# Autodesk Inventor assembly: 期末專案
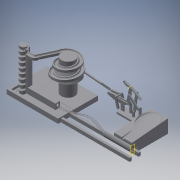
[picture p0: Inventor's stored thumbnail of the model, 180x180]
Saved by Autodesk Inventor 2017 (Build 210142000, 142)
## iProperties
Part Number: 期末專案
Material: 一般
Document SubType Name: Assembly
Designer: 士正
Author: 士正
## Documents named in this file (15)
- C:\Users\士正\Desktop\git\期末專案\期末專案.iam
- C:\Users\士正\Desktop\git\期末專案\實體1_3.ipt
- C:\Users\士正\Desktop\git\期末專案\實體2_3.ipt
- C:\Users\士正\Desktop\git\期末專案\實體3_3.ipt
- C:\Users\士正\Desktop\git\期末專案\實體4_3.ipt
- C:\Users\士正\Desktop\git\期末專案\實體5_3.ipt
- C:\Users\士正\Desktop\git\期末專案\實體6_3.ipt
- C:\Users\士正\Desktop\git\期末專案\實體7_3.ipt
- C:\Users\士正\Desktop\git\期末專案\實體8_3.ipt
- C:\Users\士正\Desktop\git\期末專案\實體9_3.ipt
- C:\Users\士正\Desktop\git\期末專案\實體10_2.ipt
- C:\Users\士正\Desktop\git\期末專案\實體11_2.ipt
- C:\Users\士正\Desktop\git\期末專案\螺旋5.ipt
- C:\Users\士正\Desktop\git\期末專案\零件2.ipt
- C:\Users\士正\Desktop\git\期末專案\長方形塊.ipt
## Components (28 placed, 14 different names)
1. 實體1_3:1 — 貼合:7, 貼合:8, 貼合:12
2. 實體2_3:1 — 貼合:11, 貼合:21, 貼合:22, 貼合:35, 齊平:11, 貼合:36, 齊平:12
3. 實體3_3:1 — 貼合:9, 貼合:10, 貼合:13, 貼合:14, 貼合:34, 齊平:10
4. 實體4_3:1 — 貼合:3, 貼合:4, 貼合:5, 貼合:6
5. 實體5_3:1 — 貼合:5, 貼合:6, 貼合:18, 貼合:29, 齊平:5
6. 實體6_3:1 — 貼合:1, 貼合:2, 貼合:17, 貼合:27, 齊平:3, 貼合:31, 齊平:7
7. 實體7_3:1 — 貼合:19, 貼合:20, 貼合:21, 貼合:22, 貼合:23, 貼合:25, 齊平:1, 貼合:37, 齊平:13, 貼合:40, 齊平:16
8. 實體8_3:1 — 貼合:12, 貼合:13, 貼合:14, 貼合:15, 貼合:16, 貼合:19, 貼合:20, 貼合:32, 齊平:8, 貼合:33, 齊平:9
9. 實體9_3:1 — 貼合:15, 貼合:16, 貼合:17, 貼合:18, 貼合:30, 齊平:6
10. 實體10_2:1 — 貼合:29, 齊平:5
11. 實體11_2:1 — 貼合:1, 貼合:2, 貼合:3, 貼合:4, 貼合:7, 貼合:8, 貼合:9, 貼合:10, 貼合:11, 貼合:24, 齊平:2, 貼合:26, 貼合:28, 齊平:4, 貼合:41, 齊平:17, 齊平:18
12. 實體2_3:2 — 貼合:23, 貼合:24, 貼合:25, 貼合:38, 齊平:14, 貼合:39, 齊平:15
13. 實體10_2:2 — 貼合:31, 齊平:7
14. 實體10_2:3 — 貼合:37, 齊平:13
15. 實體10_2:4 — 貼合:40, 齊平:16
16. 實體10_2:5 — 貼合:39, 齊平:15
17. 實體10_2:6 — 貼合:36, 齊平:12
18. 實體10_2:7 — 貼合:35, 齊平:11
19. 實體10_2:8 — 貼合:38, 齊平:14
20. 實體10_2:9 — 貼合:32, 齊平:8
21. 實體10_2:10 — 貼合:34, 齊平:10
22. 實體10_2:11 — 貼合:33, 齊平:9
23. 實體10_2:12 — 貼合:27, 齊平:3
24. 實體10_2:13 — 貼合:30, 齊平:6
25. 實體10_2:14 — 貼合:28, 齊平:4
26. 螺旋5:1 — 齊平:1, 齊平:2, 貼合:26, 齊平:21
27. 零件2:1 — 齊平:19
28. 長方形塊:1 — 齊平:20, 齊平:21
## Relationships (62: Mate 41, Flush 21)
- 貼合:1 [Mate]: 實體6_3:1 ↔ 實體11_2:1
- 貼合:2 [Mate]: 實體6_3:1 ↔ 實體11_2:1
- 貼合:3 [Mate]: 實體4_3:1 ↔ 實體11_2:1
- 貼合:4 [Mate]: 實體4_3:1 ↔ 實體11_2:1
- 貼合:5 [Mate]: 實體4_3:1 ↔ 實體5_3:1
- 貼合:6 [Mate]: 實體4_3:1 ↔ 實體5_3:1
- 貼合:7 [Mate]: 實體1_3:1 ↔ 實體11_2:1
- 貼合:8 [Mate]: 實體1_3:1 ↔ 實體11_2:1
- 貼合:9 [Mate]: 實體3_3:1 ↔ 實體11_2:1
- 貼合:10 [Mate]: 實體3_3:1 ↔ 實體11_2:1
- 貼合:11 [Mate]: 實體2_3:1 ↔ 實體11_2:1
- 貼合:12 [Mate]: 實體1_3:1 ↔ 實體8_3:1
- 貼合:13 [Mate]: 實體3_3:1 ↔ 實體8_3:1
- 貼合:14 [Mate]: 實體3_3:1 ↔ 實體8_3:1
- 貼合:15 [Mate]: 實體8_3:1 ↔ 實體9_3:1
- 貼合:16 [Mate]: 實體8_3:1 ↔ 實體9_3:1
- 貼合:17 [Mate]: 實體6_3:1 ↔ 實體9_3:1
- 貼合:18 [Mate]: 實體5_3:1 ↔ 實體9_3:1
- 貼合:19 [Mate]: 實體7_3:1 ↔ 實體8_3:1
- 貼合:20 [Mate]: 實體7_3:1 ↔ 實體8_3:1
- 貼合:21 [Mate]: 實體2_3:1 ↔ 實體7_3:1
- 貼合:22 [Mate]: 實體2_3:1 ↔ 實體7_3:1
- 貼合:23 [Mate]: 實體7_3:1 ↔ 實體2_3:2
- 貼合:24 [Mate]: 實體11_2:1 ↔ 實體2_3:2
- 貼合:25 [Mate]: 實體7_3:1 ↔ 實體2_3:2
- 齊平:1 [Flush]: 實體7_3:1 ↔ 螺旋5:1
- 齊平:2 [Flush]: 實體11_2:1 ↔ 螺旋5:1
- 貼合:26 [Mate] (93 mm): 實體11_2:1 ↔ 螺旋5:1
- 貼合:27 [Mate]: 實體6_3:1 ↔ 實體10_2:12
- 齊平:3 [Flush]: 實體6_3:1 ↔ 實體10_2:12
- 貼合:28 [Mate]: 實體11_2:1 ↔ 實體10_2:14
- 齊平:4 [Flush]: 實體11_2:1 ↔ 實體10_2:14
- 貼合:29 [Mate]: 實體5_3:1 ↔ 實體10_2:1
- 齊平:5 [Flush]: 實體5_3:1 ↔ 實體10_2:1
- 貼合:30 [Mate]: 實體9_3:1 ↔ 實體10_2:13
- 貼合:31 [Mate]: 實體6_3:1 ↔ 實體10_2:2
- 齊平:6 [Flush]: 實體9_3:1 ↔ 實體10_2:13
- 齊平:7 [Flush]: 實體6_3:1 ↔ 實體10_2:2
- 貼合:32 [Mate]: 實體8_3:1 ↔ 實體10_2:9
- 齊平:8 [Flush]: 實體8_3:1 ↔ 實體10_2:9
- 貼合:33 [Mate]: 實體8_3:1 ↔ 實體10_2:11
- 齊平:9 [Flush]: 實體8_3:1 ↔ 實體10_2:11
- 貼合:34 [Mate]: 實體3_3:1 ↔ 實體10_2:10
- 齊平:10 [Flush]: 實體3_3:1 ↔ 實體10_2:10
- 貼合:35 [Mate]: 實體2_3:1 ↔ 實體10_2:7
- 齊平:11 [Flush]: 實體2_3:1 ↔ 實體10_2:7
- 貼合:36 [Mate]: 實體2_3:1 ↔ 實體10_2:6
- 齊平:12 [Flush]: 實體2_3:1 ↔ 實體10_2:6
- 貼合:37 [Mate]: 實體7_3:1 ↔ 實體10_2:3
- 齊平:13 [Flush]: 實體7_3:1 ↔ 實體10_2:3
- 貼合:38 [Mate]: 實體2_3:2 ↔ 實體10_2:8
- 齊平:14 [Flush]: 實體2_3:2 ↔ 實體10_2:8
- 貼合:39 [Mate]: 實體2_3:2 ↔ 實體10_2:5
- 齊平:15 [Flush]: 實體2_3:2 ↔ 實體10_2:5
- 貼合:40 [Mate]: 實體7_3:1 ↔ 實體10_2:4
- 齊平:16 [Flush]: 實體7_3:1 ↔ 實體10_2:4
- 貼合:41 [Mate]: 實體11_2:1
- 齊平:17 [Flush]: 實體11_2:1
- 齊平:18 [Flush]: 實體11_2:1
- 齊平:19 [Flush]: 零件2:1
- 齊平:20 [Flush]: 長方形塊:1
- 齊平:21 [Flush]: 螺旋5:1 ↔ 長方形塊:1
